# Autodesk Inventor assembly: RemovableStageAssembly
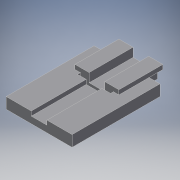
[picture p0: Inventor's stored thumbnail of the model, 180x180]
Saved by Autodesk Inventor 2019 (Build 230136000, 136)
## iProperties
Created: 2019-06-18
Part Number: RemovableStageAssembly
Document SubType Name: Assembly
Designer: aorfi
Author: aorfi
## Documents named in this file (3)
- C:\Users\aorfi\Documents\IQC\RemovableStageAssembly.iam
- C:\Users\aorfi\Documents\IQC\CustomParts\RS-FixedFiber.ipt
- C:\Users\aorfi\Documents\IQC\CustomParts\RS-RemovableFiber.ipt
## Components (2 placed, 2 different names)
1. RS-RemovableFiber:1 — Flush:1, Flush:2, Flush:3, Flush:4, Mate:1
2. RS-FixedFiber:1 — Flush:4, Mate:1
## Relationships (5: Flush 4, Mate 1)
- Flush:1: RS-RemovableFiber:1
- Flush:2: RS-RemovableFiber:1
- Flush:3: RS-RemovableFiber:1
- Flush:4: RS-RemovableFiber:1 ↔ RS-FixedFiber:1
- Mate:1: RS-RemovableFiber:1 ↔ RS-FixedFiber:1
